# Autodesk Inventor assembly: CL-4-F
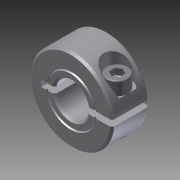
[picture p0: Inventor's stored thumbnail of the model, 180x180]
Saved by Autodesk Inventor 2012 (Build 160160000, 160)
## iProperties
Category: Miscellaneous
Company: Autodesk Inc.
Created: 2011-11-15
Part Number: CL-4-F
Document SubType Name: Assembly
Designer: Autodesk Inc.
Catalog Web Link: http://www.ruland.com/ps_collars_shaft_cl.asp
Description: 1/4 " ID 1/2" OD Clamp Shaft Collar
Vendor: Ruland Manufacturing
Author: Autodesk Inc.
## Documents named in this file (3)
- C:\Data Folder\FIRST 2012\KOP\All Parts 2012\Miscellaneous\Misc_ShaftCollar_Ruland_CL-4-F.iam
- C:\Data Folder\FIRST 2012\KOP\All Parts 2012\Miscellaneous\Misc_Collars_Ruland_CL-4-F.ipt
- C:\Data Folder\FIRST 2012\KOP\All Parts 2012\Miscellaneous\ANSI B18.3 - 3-48 UNC - 0.25(31).ipt
## Components (2 placed, 2 different names)
1. Misc_Collars_Ruland_CL-4-F:1 — Insert:1
2. Hexagon Socket Head Cap Screw - Inch No. 3 - 48 UNC - 1/4:1 — Insert:1
## Relationships (1: Insert 1)
- Insert:1: Misc_Collars_Ruland_CL-4-F:1 ↔ Hexagon Socket Head Cap Screw - Inch No. 3 - 48 UNC - 1/4:1
